# Autodesk Inventor assembly: encoder_todo_junto
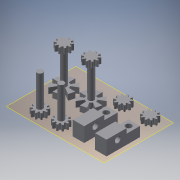
[picture p0: Inventor's stored thumbnail of the model, 180x180]
Saved by Autodesk Inventor 2019 (Build 230136000, 136)
## iProperties
Created: 2018-11-27
Part Number: encoder_todo_junto
Document SubType Name: Assembly
Designer: Andres
Author: Andres
## Documents named in this file (5)
- C:\Users\Andres\Documents\GitHub\Shank2.0\Variados\Diseño Mecanico\encoder_todo_junto.iam
- C:\Users\Andres\Documents\GitHub\Shank2.0\Variados\Diseño Mecanico\encoder_engranaje.ipt
- C:\Users\Andres\Documents\GitHub\Shank2.0\Variados\Diseño Mecanico\EncoderBase.ipt
- C:\Users\Andres\Documents\GitHub\Shank2.0\Variados\Diseño Mecanico\encoder_engranaje_separado.ipt
- C:\Users\Andres\Documents\GitHub\Shank2.0\Variados\Diseño Mecanico\encoder_engranaje_separado2.ipt
## Components (8 placed, 4 different names)
1. encoder_engranaje:1 — Mate:3
2. EncoderBase:1 — Mate:1
3. encoder_engranaje:2 — Mate:4
4. EncoderBase:2 — Mate:2
5. encoder_engranaje_separado:1 — Mate:8
6. encoder_engranaje_separado2:1 — Mate:6
7. encoder_engranaje_separado:2 — Mate:7
8. encoder_engranaje_separado2:2 — Mate:5
## Relationships (8: Mate 8)
- Mate:1: EncoderBase:1
- Mate:2: EncoderBase:2
- Mate:3: encoder_engranaje:1
- Mate:4: encoder_engranaje:2
- Mate:5: encoder_engranaje_separado2:2
- Mate:6: encoder_engranaje_separado2:1
- Mate:7: encoder_engranaje_separado:2
- Mate:8: encoder_engranaje_separado:1
